# Autodesk Inventor assembly: LEG1
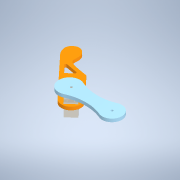
[picture p0: Inventor's stored thumbnail of the model, 180x180]
Saved by Autodesk Inventor 2020.3 (Build 243373000, 373)
## iProperties
Created: 2020-08-08
Part Number: LEG1
Document SubType Name: Assembly
Designer: aditk
Author: aditk
## Documents named in this file (4)
- C:\Users\aditk\Desktop\newCat\LEG1.iam
- C:\Users\aditk\Desktop\newCat\big_servo.ipt
- C:\Users\aditk\Desktop\newCat\leg2.ipt
- C:\Users\aditk\Desktop\newCat\thai.ipt
## Components (3 placed, 3 different names)
1. big_servo:1 — Mate:1, Mate:2, Mate:3, Insert:1
2. leg2:1 — Mate:1, Mate:2, Mate:3
3. thai:1 — Insert:1
## Relationships (4: Mate 3, Insert 1)
- Mate:1: big_servo:1 ↔ leg2:1
- Mate:2: big_servo:1 ↔ leg2:1
- Mate:3: big_servo:1 ↔ leg2:1
- Insert:1 (0.254 mm): big_servo:1 ↔ thai:1
